# Autodesk Inventor assembly: Assembly servo2
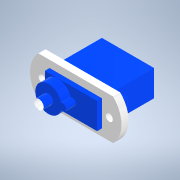
[picture p0: Inventor's stored thumbnail of the model, 180x180]
Saved by Autodesk Inventor 2021 (Build 250183000, 183)
## iProperties
Created: 2023-06-06
Part Number: Assembly servo2
Document SubType Name: Assembly
Designer: shrus
Author: shrus
## Documents named in this file (3)
- C:\Users\shrus\Documents\Assembly servo2.iam
- C:\Users\shrus\Documents\servo1.ipt
- C:\Users\shrus\Documents\servo Holder.ipt
## Components (2 placed, 2 different names)
1. servo1:1 — Mate:1, Mate:2, Mate:3
2. servo Holder:1 — Mate:1, Mate:2, Mate:3
## Relationships (3: Mate 3)
- Mate:1: servo1:1 ↔ servo Holder:1
- Mate:2: servo1:1 ↔ servo Holder:1
- Mate:3: servo1:1 ↔ servo Holder:1
